# Autodesk Inventor assembly: xy mount
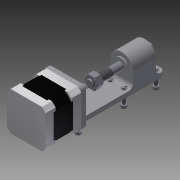
[picture p0: Inventor's stored thumbnail of the model, 180x180]
Saved by Autodesk Inventor 2014 (Build 180170000, 170)
## iProperties
Created: 2013-10-14
Part Number: xy mount
Document SubType Name: Assembly
Designer: employee
Author: employee
## Documents named in this file (9)
- \\GRISTLE\speco\GitHub\ConceptFORGE\Wally\xy mount.iam
- \\GRISTLE\speco\GitHub\ConceptFORGE\Wally\xy mount.ipt
- \\GRISTLE\speco\GitHub\ConceptFORGE\Wally\M3x10.ipt
- \\GRISTLE\speco\GitHub\ConceptFORGE\Wally\m3 nut.ipt
- \\GRISTLE\speco\GitHub\ConceptFORGE\Wally\M3x16.ipt
- \\GRISTLE\speco\GitHub\ConceptFORGE\Wally\stepper.ipt
- \\GRISTLE\speco\GitHub\ConceptFORGE\Wally\M8x60.ipt
- \\GRISTLE\speco\GitHub\ConceptFORGE\Wally\washer.ipt
- \\GRISTLE\speco\GitHub\ConceptFORGE\Wally\M8 nut.ipt
## Components (21 placed, 8 different names)
1. xy mount:1 — Insert:1, Insert:2, Insert:3, Insert:4, Angle:1, Angle:2, Angle:3, Angle:4, Angle:5, Angle:6, Insert:5, Insert:6, Insert:7, Insert:8, Insert:9, Insert:10, Insert:11, Insert:12, Insert:13, Insert:14, Insert:15, Insert:16, Insert:17, Angle:7, Insert:18, Insert:19
2. M3x10:1 — Insert:3
3. M3x10:2 — Insert:4
4. M3x10:3 — Insert:1
5. M3x10:4 — Insert:2
6. Hex Nut Metric M3 x 0.5:1 — Angle:1, Insert:5
7. Hex Nut Metric M3 x 0.5:2 — Angle:2, Insert:10
8. Hex Nut Metric M3 x 0.5:3 — Angle:3, Insert:7
9. Hex Nut Metric M3 x 0.5:4 — Angle:4, Insert:8
10. Hex Nut Metric M3 x 0.5:5 — Angle:6, Insert:6
11. Hex Nut Metric M3 x 0.5:6 — Angle:5, Insert:9
12. Forged Socket Head Cap Screw - Metric M3x0.5 x 16:1 — Insert:11
13. Forged Socket Head Cap Screw - Metric M3x0.5 x 16:2 — Insert:12
14. Forged Socket Head Cap Screw - Metric M3x0.5 x 16:3 — Insert:13
15. Forged Socket Head Cap Screw - Metric M3x0.5 x 16:4 — Insert:14
16. Forged Socket Head Cap Screw - Metric M3x0.5 x 16:5 — Insert:15
17. Forged Socket Head Cap Screw - Metric M3x0.5 x 16:6 — Insert:16
18. stepper:1 — Insert:17, Angle:7
19. Hex Bolt - Metric M8 x 1.25 x 60:1 — Insert:18
20. washer:1 — Insert:19, Insert:20
21. Hex Nut Metric M8 x 1.25:1 — Insert:20
## Relationships (27: Insert 20, Angle 7)
- Insert:1: xy mount:1 ↔ M3x10:3
- Insert:2: xy mount:1 ↔ M3x10:4
- Insert:3: xy mount:1 ↔ M3x10:1
- Insert:4: xy mount:1 ↔ M3x10:2
- Angle:1 (0 deg): xy mount:1 ↔ Hex Nut Metric M3 x 0.5:1
- Angle:2 (0 deg): xy mount:1 ↔ Hex Nut Metric M3 x 0.5:2
- Angle:3 (0 deg): xy mount:1 ↔ Hex Nut Metric M3 x 0.5:3
- Angle:4 (0 deg): xy mount:1 ↔ Hex Nut Metric M3 x 0.5:4
- Angle:5 (0 deg): xy mount:1 ↔ Hex Nut Metric M3 x 0.5:6
- Angle:6 (0 deg): xy mount:1 ↔ Hex Nut Metric M3 x 0.5:5
- Insert:5: xy mount:1 ↔ Hex Nut Metric M3 x 0.5:1
- Insert:6: xy mount:1 ↔ Hex Nut Metric M3 x 0.5:5
- Insert:7: xy mount:1 ↔ Hex Nut Metric M3 x 0.5:3
- Insert:8: xy mount:1 ↔ Hex Nut Metric M3 x 0.5:4
- Insert:9: xy mount:1 ↔ Hex Nut Metric M3 x 0.5:6
- Insert:10: xy mount:1 ↔ Hex Nut Metric M3 x 0.5:2
- Insert:11 (9.5 mm): xy mount:1 ↔ Forged Socket Head Cap Screw - Metric M3x0.5 x 16:1
- Insert:12 (9.5 mm): xy mount:1 ↔ Forged Socket Head Cap Screw - Metric M3x0.5 x 16:2
- Insert:13 (9.5 mm): xy mount:1 ↔ Forged Socket Head Cap Screw - Metric M3x0.5 x 16:3
- Insert:14 (9.5 mm): xy mount:1 ↔ Forged Socket Head Cap Screw - Metric M3x0.5 x 16:4
- Insert:15 (9.5 mm): xy mount:1 ↔ Forged Socket Head Cap Screw - Metric M3x0.5 x 16:5
- Insert:16 (9.5 mm): xy mount:1 ↔ Forged Socket Head Cap Screw - Metric M3x0.5 x 16:6
- Insert:17: xy mount:1 ↔ stepper:1
- Angle:7 (0 deg): xy mount:1 ↔ stepper:1
- Insert:18: xy mount:1 ↔ Hex Bolt - Metric M8 x 1.25 x 60:1
- Insert:19: xy mount:1 ↔ washer:1
- Insert:20 (25 mm): washer:1 ↔ Hex Nut Metric M8 x 1.25:1
